# Autodesk Inventor assembly: FullRobotAssembly
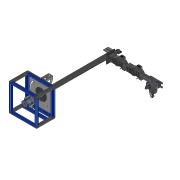
[picture p0: Inventor's stored thumbnail of the model, 180x180]
Saved by Autodesk Inventor 2020.3 (Build 243373000, 373)
## iProperties
Created: 2021-08-04
Part Number: FullRobotAssembly
Document SubType Name: Assembly
Designer: justi
Author: justi
## Documents named in this file (10)
- F:\UQ Engineering\2021 ~ 5th Year\Semester 2\METR4911-THESIS\FarmBot CAD\FarmBotV1\FullRobotAssembly.iam
- F:\UQ Engineering\2021 ~ 5th Year\Semester 2\METR4911-THESIS\FarmBot CAD\FarmBotV1\VerticalAssembly.iam
- F:\UQ Engineering\2021 ~ 5th Year\Semester 2\METR4911-THESIS\FarmBot CAD\FarmBotV1\CycloidalJoint1.iam
- F:\UQ Engineering\2021 ~ 5th Year\Semester 2\METR4911-THESIS\FarmBot CAD\FarmBotV1\BaseAssembly_V2.iam
- F:\UQ Engineering\2021 ~ 5th Year\Semester 2\METR4911-THESIS\FarmBot CAD\FarmBotV1\FullRobotAssembly\AIP\FEA\dpg72ywsg.fins
- F:\UQ Engineering\2021 ~ 5th Year\Semester 2\METR4911-THESIS\FarmBot CAD\FarmBotV1\FullRobotAssembly\AIP\FEA\dpg72ywtc.fsat
- F:\UQ Engineering\2021 ~ 5th Year\Semester 2\METR4911-THESIS\FarmBot CAD\FarmBotV1\FullRobotAssembly\AIP\FEA\dpg72ywtc.ftes
- F:\UQ Engineering\2021 ~ 5th Year\Semester 2\METR4911-THESIS\FarmBot CAD\FarmBotV1\FullRobotAssembly\AIP\FEA\dpg72ywtc.fwiz
- F:\UQ Engineering\2021 ~ 5th Year\Semester 2\METR4911-THESIS\FarmBot CAD\FarmBotV1\FullRobotAssembly\AIP\FEA\dpg72yxfk.fmsh
- F:\UQ Engineering\2021 ~ 5th Year\Semester 2\METR4911-THESIS\FarmBot CAD\FarmBotV1\FullRobotAssembly\AIP\FEA\dpg72yxgg.fres
## Components (3 placed, 3 different names)
1. VerticalAssembly:1 [sub-assembly] — Mate:3, Mate:4, Mate:5, Mate:11, Mate:12
2. CycloidalJoint1:1 [sub-assembly] — Mate:3, Mate:4, Mate:5
3. BaseAssembly_V2:1 [sub-assembly] — Mate:11, Mate:12, Mate:13, Flush:1
## Relationships (7: Mate 6, Flush 1)
- Mate:3: VerticalAssembly:1 ↔ CycloidalJoint1:1
- Mate:4: VerticalAssembly:1 ↔ CycloidalJoint1:1
- Mate:5: VerticalAssembly:1 ↔ CycloidalJoint1:1
- Mate:11: VerticalAssembly:1 ↔ BaseAssembly_V2:1
- Mate:12: VerticalAssembly:1 ↔ BaseAssembly_V2:1
- Mate:13: BaseAssembly_V2:1
- Flush:1: BaseAssembly_V2:1
## Named parameters: sa_0 = 981, sa_1 = 98100
note: some values were not read from the file. Shown as the stored number, unit unknown: "sa_0", "sa_1".
